# Autodesk Inventor assembly: 4x2020_subaxis-asm
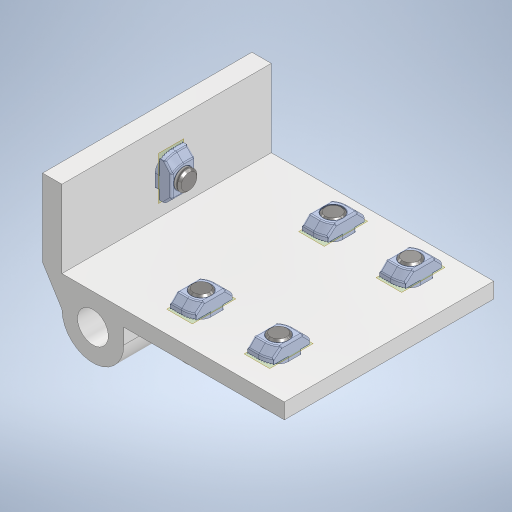
[picture p0: Inventor's stored thumbnail of the model, 512x512]
Saved by Autodesk Inventor 2024 (Build 280153000, 153)
## iProperties
Created: 2025-12-25
Part Number: 4x2020_subaxis-asm
Document SubType Name: Assembly
Designer: schar
Author: schar
## Documents named in this file (6)
- C:\Users\schar\Desktop\projectBlueprint\AMSTS\hardware\4x2020_subaxis-asm.iam
- C:\Users\schar\Desktop\projectBlueprint\AMSTS\hardware\4x2020_subaxis.ipt
- C:\Users\schar\Documents\Inventor\Content Center Files\R2024\en-US\DIN 9021\DIN 9021 - 5,3.ipt
- C:\Users\schar\Desktop\projectBlueprint\AMSTS\hardware\tnut_m5_2020.ipt
- C:\Users\schar\Documents\Inventor\Content Center Files\R2024\en-US\ISO 4762(1)\DIN EN ISO 4762 - M5 x 10.ipt
- C:\Users\schar\Documents\Inventor\Content Center Files\R2024\en-US\ISO 4762(1)\DIN EN ISO 4762 - M5 x 12.ipt
## Components (16 placed, 5 different names)
1. 4x2020_subaxis:1 — Mate:1, Mate:2, Mate:3, Mate:4, Mate:5, Mate:6, Mate:7, Mate:8, Mate:9, Mate:10, Rigid:6, Rigid:5, Rigid:4, Rigid:1, Rigid:7, Mate:22
2. DIN 9021 5,3:1 — Mate:2, Mate:9, Mate:13, Mate:21
3. DIN 9021 5,3:2 — Mate:1, Mate:7, Mate:12, Mate:17
4. DIN 9021 5,3:3 — Mate:3, Mate:10, Mate:14, Mate:20
5. DIN 9021 5,3:4 — Mate:4, Mate:8, Mate:11, Mate:19
6. DIN 9021 5,3:5 — Mate:5, Mate:6, Mate:23
7. tnut_m5_2020:1 — Rigid:7
8. tnut_m5_2020:2 — Rigid:1
9. tnut_m5_2020:3 — Rigid:4
10. tnut_m5_2020:4 — Rigid:5
11. tnut_m5_2020:5 — Rigid:6
12. DIN EN ISO 4762 M5 x 10:2 — Mate:12, Mate:17
13. DIN EN ISO 4762 M5 x 10:3 — Mate:11, Mate:19
14. DIN EN ISO 4762 M5 x 10:4 — Mate:13, Mate:21
15. DIN EN ISO 4762 M5 x 10:5 — Mate:14, Mate:20
16. DIN EN ISO 4762 M5 x 12:1 — Mate:22, Mate:23
## Relationships (25: Mate 20, WeldJoint 5)
- Mate:1: 4x2020_subaxis:1 ↔ DIN 9021 5,3:2
- Mate:2: 4x2020_subaxis:1 ↔ DIN 9021 5,3:1
- Mate:3: 4x2020_subaxis:1 ↔ DIN 9021 5,3:3
- Mate:4: 4x2020_subaxis:1 ↔ DIN 9021 5,3:4
- Mate:5: 4x2020_subaxis:1 ↔ DIN 9021 5,3:5
- Mate:6: 4x2020_subaxis:1 ↔ DIN 9021 5,3:5
- Mate:7: 4x2020_subaxis:1 ↔ DIN 9021 5,3:2
- Mate:8: 4x2020_subaxis:1 ↔ DIN 9021 5,3:4
- Mate:9: 4x2020_subaxis:1 ↔ DIN 9021 5,3:1
- Mate:10: 4x2020_subaxis:1 ↔ DIN 9021 5,3:3
- Rigid:6 [WeldJoint] (0.159 mm): 4x2020_subaxis:1 ↔ tnut_m5_2020:5
- Rigid:5 [WeldJoint] (0.159 mm): 4x2020_subaxis:1 ↔ tnut_m5_2020:4
- Rigid:4 [WeldJoint] (0.159 mm): 4x2020_subaxis:1 ↔ tnut_m5_2020:3
- Rigid:1 [WeldJoint] (0.159 mm): 4x2020_subaxis:1 ↔ tnut_m5_2020:2
- Rigid:7 [WeldJoint] (0.159 mm): 4x2020_subaxis:1 ↔ tnut_m5_2020:1
- Mate:11: DIN 9021 5,3:4 ↔ DIN EN ISO 4762 M5 x 10:3
- Mate:12: DIN 9021 5,3:2 ↔ DIN EN ISO 4762 M5 x 10:2
- Mate:13: DIN 9021 5,3:1 ↔ DIN EN ISO 4762 M5 x 10:4
- Mate:14: DIN 9021 5,3:3 ↔ DIN EN ISO 4762 M5 x 10:5
- Mate:17: DIN 9021 5,3:2 ↔ DIN EN ISO 4762 M5 x 10:2
- Mate:19: DIN 9021 5,3:4 ↔ DIN EN ISO 4762 M5 x 10:3
- Mate:20: DIN 9021 5,3:3 ↔ DIN EN ISO 4762 M5 x 10:5
- Mate:21: DIN 9021 5,3:1 ↔ DIN EN ISO 4762 M5 x 10:4
- Mate:22: 4x2020_subaxis:1 ↔ DIN EN ISO 4762 M5 x 12:1
- Mate:23: DIN 9021 5,3:5 ↔ DIN EN ISO 4762 M5 x 12:1
